# Autodesk Inventor assembly: Todo
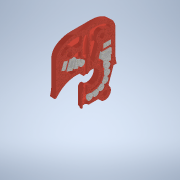
[picture p0: Inventor's stored thumbnail of the model, 180x180]
Saved by Autodesk Inventor 2021 (Build 250183000, 183)
## iProperties
Created: 2021-08-28
Part Number: Todo
Document SubType Name: Assembly
Designer: Diego.labarca
Author: Diego.labarca
## Documents named in this file (5)
- E:\Dropbox\Inventor\Impresora 3D\Arreglos Impresora\Mini AB Sensors\Todo.iam
- E:\Dropbox\Inventor\Impresora 3D\Arreglos Impresora\Mini AB Sensors\Iman 5x3.ipt
- E:\Dropbox\Inventor\Impresora 3D\Arreglos Impresora\Mini AB Sensors\Ball 4mm.ipt
- E:\Dropbox\Inventor\Impresora 3D\Arreglos Impresora\Mini AB Sensors\Sensores.ipt
- E:\Dropbox\Inventor\Impresora 3D\Arreglos Impresora\Mini AB Sensors\Porta Hall Sensor.ipt
## Components (14 placed, 4 different names)
1. Sensores:1 — Coincidencia:1, Nivelación:8, Coincidencia:3, Coincidencia:4, Coincidencia:6, Coincidencia:7, Coincidencia:8, Coincidencia:10, Nivelación:14, Coincidencia:11, Coincidencia:12, Coincidencia:13, Coincidencia:14
2. Iman 5x3:1 — Tangente:6, Coincidencia:3, Coincidencia:9
3. Ball 4mm:1 — Coincidencia:1, Nivelación:8, Ángulo:1, Nivelación:9, Tangente:1, Nivelación:10, Nivelación:11, Nivelación:12, Nivelación:13
4. Ball 4mm:2 — Nivelación:9, Tangente:1, Tangente:2
5. Ball 4mm:3 — Nivelación:10, Tangente:2, Tangente:3
6. Ball 4mm:4 — Nivelación:11, Tangente:3, Tangente:4
7. Ball 4mm:5 — Nivelación:12, Tangente:4, Tangente:5
8. Ball 4mm:6 — Nivelación:13, Tangente:5, Tangente:6
9. Ball 4mm:7 — Coincidencia:4, Tangente:7
10. Iman 5x3:2 — Coincidencia:6, Tangente:7
11. Iman 5x3:3 — Coincidencia:7, Coincidencia:8
12. Iman 5x3:4 — Coincidencia:9, Coincidencia:10
13. Porta Hall Sensor:1 — Nivelación:14, Coincidencia:11, Coincidencia:12, Nivelación:15
14. Porta Hall Sensor:2 — Nivelación:15, Coincidencia:13, Coincidencia:14
## Relationships (28: Mate 12, Flush 8, Tangent 7, Angle 1)
- Coincidencia:1 [Mate]: Sensores:1 ↔ Ball 4mm:1
- Nivelación:8 [Flush] (-2.875 mm): Sensores:1 ↔ Ball 4mm:1
- Ángulo:1 [Angle] (0 deg): Ball 4mm:1
- Nivelación:9 [Flush]: Ball 4mm:1 ↔ Ball 4mm:2
- Tangente:1: Ball 4mm:1 ↔ Ball 4mm:2
- Nivelación:10 [Flush]: Ball 4mm:1 ↔ Ball 4mm:3
- Tangente:2: Ball 4mm:2 ↔ Ball 4mm:3
- Nivelación:11 [Flush]: Ball 4mm:1 ↔ Ball 4mm:4
- Tangente:3: Ball 4mm:3 ↔ Ball 4mm:4
- Nivelación:12 [Flush]: Ball 4mm:1 ↔ Ball 4mm:5
- Tangente:4: Ball 4mm:4 ↔ Ball 4mm:5
- Nivelación:13 [Flush]: Ball 4mm:1 ↔ Ball 4mm:6
- Tangente:5: Ball 4mm:5 ↔ Ball 4mm:6
- Tangente:6: Iman 5x3:1 ↔ Ball 4mm:6
- Coincidencia:3 [Mate]: Sensores:1 ↔ Iman 5x3:1
- Coincidencia:4 [Mate]: Sensores:1 ↔ Ball 4mm:7
- Coincidencia:6 [Mate]: Sensores:1 ↔ Iman 5x3:2
- Tangente:7: Ball 4mm:7 ↔ Iman 5x3:2
- Coincidencia:7 [Mate]: Sensores:1 ↔ Iman 5x3:3
- Coincidencia:8 [Mate]: Sensores:1 ↔ Iman 5x3:3
- Coincidencia:9 [Mate]: Iman 5x3:1 ↔ Iman 5x3:4
- Coincidencia:10 [Mate]: Sensores:1 ↔ Iman 5x3:4
- Nivelación:14 [Flush]: Sensores:1 ↔ Porta Hall Sensor:1
- Coincidencia:11 [Mate]: Sensores:1 ↔ Porta Hall Sensor:1
- Coincidencia:12 [Mate]: Sensores:1 ↔ Porta Hall Sensor:1
- Nivelación:15 [Flush]: Porta Hall Sensor:1 ↔ Porta Hall Sensor:2
- Coincidencia:13 [Mate]: Sensores:1 ↔ Porta Hall Sensor:2
- Coincidencia:14 [Mate]: Sensores:1 ↔ Porta Hall Sensor:2
